# Autodesk Inventor assembly: robot
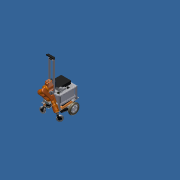
[picture p0: Inventor's stored thumbnail of the model, 180x180]
Saved by Autodesk Inventor 2012 (Build 160160000, 160)
## iProperties
Created: 2012-03-08
Part Number: robot
Document SubType Name: Assembly
Designer: esv
Mass: 169922 g
Surface Area: 87342.5 cm^2
Volume: 147894 cm^3
Density: 1.14894 g/cm^3
Author: esv
## Documents named in this file (28)
- C:\Users\Edward\Documents\masters\CAD\robot.iam
- C:\Users\Edward\Documents\masters\CAD\Frame\frame bracket.ipt
- C:\Users\Edward\Documents\masters\CAD\Invacare\invacare assy.iam
- C:\Users\Edward\Documents\masters\CAD\IRC5\IRC5_Compact.ipt
- C:\Users\Edward\Documents\masters\CAD\Frame\lower side rail.ipt
- C:\Users\Edward\Documents\masters\CAD\Frame\lower front rail.ipt
- C:\Users\Edward\Documents\masters\CAD\Frame\lower vertical rail.ipt
- C:\Users\Edward\Documents\masters\CAD\PC\PC.ipt
- C:\Users\Edward\Documents\masters\CAD\SICK\SICK LMS291.ipt
- C:\Users\Edward\Documents\masters\CAD\Frame\arm rail.ipt
- C:\Users\Edward\Documents\masters\CAD\IRB120\IRB120.iam
- C:\Users\Edward\Documents\masters\CAD\Frame\front upright.ipt
- C:\Users\Edward\Documents\masters\CAD\Kinect\Kinect.ipt
- C:\Users\Edward\Documents\masters\CAD\Frame\front top side rail.ipt
- C:\Users\Edward\Documents\masters\CAD\Frame\aim rail cross brace.ipt
- C:\Users\Edward\Documents\masters\CAD\Frame\back frame plate.ipt
- C:\Users\Edward\Documents\masters\CAD\Frame\front frame plate.ipt
- C:\Users\Edward\Documents\masters\CAD\Frame\top plate.ipt
- C:\Users\Edward\Documents\masters\CAD\Pneumatics\compressor\compressor.iam
- C:\Users\Edward\Documents\masters\CAD\Spike\Spike H.iam
- C:\Users\Edward\Documents\masters\CAD\Breaker\Breaker.iam
- C:\Users\Edward\Documents\masters\CAD\Router\router keepout.ipt
- C:\Users\Edward\Documents\masters\CAD\LIDAR Power Supply\LIDAR PSU.ipt
- C:\Users\Edward\Documents\masters\CAD\Frame\front right plate.ipt
- C:\Users\Edward\Documents\masters\CAD\Frame\front left plate.ipt
- C:\Users\Edward\Documents\masters\CAD\Frame\short frame bracket.ipt
- C:\Users\Edward\Documents\masters\CAD\base plate.iam
- C:\Users\Edward\Documents\masters\CAD\SICK\LIDAR Bracket.ipt
## Components (40 placed, 27 different names)
1. frame bracket:1 — Angle:1, Flush:5, Mate:39, Mate:40, Mate:41, Mate:72, Flush:56, Mate:74
2. frame bracket:4 — Flush:5, Mate:27, Mate:42, Mate:43, Mate:44, Flush:57, Mate:75, Mate:76
3. invacare assy:1 [sub-assembly] — Angle:1, Flush:31, Mate:18, Mate:17, Mate:68, Mate:71, Flush:54, Mate:73, Mate:77, Flush:83
4. IRC5_Compact:1 — Flush:2, Mate:7, Mate:8, Mate:99
5. lower side rail:1 — Flush:9, Flush:12, Flush:14, Flush:76, Mate:108, Mate:113, Flush:84
6. lower side rail:2 — Flush:9, Mate:6, Flush:10, Flush:12, Flush:13, Flush:41, Flush:42, Mate:45, Flush:59, Flush:62, Flush:81
7. lower side rail:3 — Flush:8, Mate:6, Flush:11, Flush:14, Mate:7, Mate:8, Flush:71
8. lower side rail:4 — Flush:8, Flush:10, Flush:11, Flush:13, Mate:79, Angle:3
9. PC:1 — Mate:36, Flush:62, Flush:63
10. SICK LMS291:1 — Insert:8, Insert:9, Mate:118
11. arm rail:1 — Flush:26, Flush:35, Mate:27, Mate:37, Tangent:1, Mate:49, Mate:53
12. arm rail:2 — Flush:26, Flush:35, Mate:30, Mate:50, Flush:49, Flush:50, Mate:84, Flush:65, Mate:115
13. IRB120:1 [sub-assembly] — Tangent:1, Mate:30, Mate:37
14. front upright:1 — Mate:39, Mate:40, Mate:41, Flush:41, Flush:42, Mate:45, Mate:47, Flush:46, Flush:47, Mate:51, Mate:101, Flush:78
15. front upright:2 — Mate:42, Mate:43, Mate:44, Flush:43, Flush:44, Flush:45, Mate:52, Flush:71, Mate:103, Flush:79
16. lower front rail:3 — Mate:47, Flush:43, Mate:112, Mate:114, Flush:84, Mate:115, Mate:116, Mate:117
17. Kinect:1 — Mate:54, Flush:51, Mate:55, Angle:2
18. front top side rail:1 — Flush:46, Flush:47, Mate:50, Mate:51, Flush:55
19. front top side rail:2 — Mate:49, Flush:44, Flush:45, Mate:52, Flush:55, Flush:77
20. aim rail cross brace:1 — Flush:49, Flush:50, Mate:53, Mate:54, Flush:51
21. back frame plate:1 — Mate:68, Flush:54, Flush:82, Insert:7
22. back frame plate:2 — Mate:71, Insert:6
23. front frame plate:1 — Flush:57, Mate:75, Mate:76, Mate:77
24. front frame plate:2 — Mate:72, Flush:56, Mate:73, Mate:74
25. top plate:1 — Mate:79, Flush:59, Mate:36, Mate:80, Flush:63, Mate:81, Insert:1, Insert:2, Insert:3, Mate:82, Insert:4, Insert:5, Flush:64, Flush:77, Mate:102
26. compressor:1 [sub-assembly] — Mate:80, Insert:2, Insert:3
27. Spike H:1 [sub-assembly] — Mate:81, Insert:1
28. Breaker:1 [sub-assembly] — Mate:82, Insert:4, Angle:3, Insert:5
29. router keepout:1 — Flush:64, Mate:83, Mate:84
30. LIDAR PSU:1 — Flush:65, Tangent:5, Tangent:6
31. lower vertical rail:1 — Flush:69, Flush:70, Flush:74, Flush:75, Mate:100, Mate:110, Mate:111
32. lower vertical rail:2 — Flush:69, Flush:70, Mate:99, Mate:104, Mate:105, Mate:106, Mate:107, Mate:108, Flush:81
33. lower front rail:4 — Flush:72, Flush:73, Flush:74, Flush:75, Mate:100
34. lower front rail:5 — Flush:72, Flush:73, Flush:76, Mate:107, Mate:109
35. front right plate:1 — Mate:101, Flush:78, Mate:102, Flush:80, Tangent:5, Tangent:6
36. front left plate:1 — Mate:103, Flush:79, Flush:80
37. short frame bracket:1 — Mate:104, Mate:105, Insert:6, Mate:106, Mate:109
38. short frame bracket:2 — Mate:110, Mate:111, Flush:82, Insert:7, Flush:83
39. base plate:1 [sub-assembly] — Mate:112, Mate:113, Mate:114
40. LIDAR Bracket:1 — Insert:8, Insert:9, Mate:116, Mate:117
## Relationships (122: Mate 59, Flush 48, Insert 9, Angle 3, Tangent 3)
- Flush:2 (-225 mm): IRC5_Compact:1
- Angle:1 (0 deg): frame bracket:1 ↔ invacare assy:1
- Flush:5: frame bracket:1 ↔ frame bracket:4
- Flush:8: lower side rail:3 ↔ lower side rail:4
- Flush:9: lower side rail:1 ↔ lower side rail:2
- Mate:6 (450.85 mm): lower side rail:2 ↔ lower side rail:3
- Flush:10: lower side rail:2 ↔ lower side rail:4
- Flush:11: lower side rail:3 ↔ lower side rail:4
- Flush:12: lower side rail:1 ↔ lower side rail:2
- Flush:13: lower side rail:2 ↔ lower side rail:4
- Flush:14: lower side rail:1 ↔ lower side rail:3
- Mate:7: IRC5_Compact:1 ↔ lower side rail:3
- Mate:8 (6.35 mm): IRC5_Compact:1 ↔ lower side rail:3
- Flush:31: invacare assy:1
- Mate:17: invacare assy:1
- Mate:18: invacare assy:1
- Flush:26: arm rail:1 ↔ arm rail:2
- Flush:35: arm rail:1 ↔ arm rail:2
- Mate:27: frame bracket:4 ↔ arm rail:1
- Tangent:1: arm rail:1 ↔ IRB120:1
- Mate:30: arm rail:2 ↔ IRB120:1
- Mate:37 (-609.6 mm): arm rail:1 ↔ IRB120:1
- Mate:36: PC:1 ↔ top plate:1
- Flush:40 (-368.3 mm)
- Mate:39: frame bracket:1 ↔ front upright:1
- Mate:40: frame bracket:1 ↔ front upright:1
- Mate:41: frame bracket:1 ↔ front upright:1
- Mate:42: frame bracket:4 ↔ front upright:2
- Mate:43: frame bracket:4 ↔ front upright:2
- Mate:44: frame bracket:4 ↔ front upright:2
- Flush:41: lower side rail:2 ↔ front upright:1
- Flush:42: lower side rail:2 ↔ front upright:1
- Mate:45: lower side rail:2 ↔ front upright:1
- Mate:47: front upright:1 ↔ lower front rail:3
- Flush:43: front upright:2 ↔ lower front rail:3
- Mate:49: arm rail:1 ↔ front top side rail:2
- Flush:44: front upright:2 ↔ front top side rail:2
- Flush:45: front upright:2 ↔ front top side rail:2
- Flush:46: front upright:1 ↔ front top side rail:1
- Flush:47: front upright:1 ↔ front top side rail:1
- Mate:50: arm rail:2 ↔ front top side rail:1
- Mate:51: front upright:1 ↔ front top side rail:1
- Mate:52: front upright:2 ↔ front top side rail:2
- Flush:49: arm rail:2 ↔ aim rail cross brace:1
- Flush:50: arm rail:2 ↔ aim rail cross brace:1
- Mate:53: arm rail:1 ↔ aim rail cross brace:1
- Mate:54: Kinect:1 ↔ aim rail cross brace:1
- Flush:51: Kinect:1 ↔ aim rail cross brace:1
- Mate:55: Kinect:1
- Angle:2 (0 deg): Kinect:1
- Mate:56
- Mate:68: invacare assy:1 ↔ back frame plate:1
- Mate:71: invacare assy:1 ↔ back frame plate:2
- Flush:54: invacare assy:1 ↔ back frame plate:1
- Flush:55: front top side rail:1 ↔ front top side rail:2
- Mate:72: frame bracket:1 ↔ front frame plate:2
- Flush:56: frame bracket:1 ↔ front frame plate:2
- Mate:73: invacare assy:1 ↔ front frame plate:2
- Mate:74: frame bracket:1 ↔ front frame plate:2
- Flush:57: frame bracket:4 ↔ front frame plate:1
- Mate:75: frame bracket:4 ↔ front frame plate:1
- Mate:76: frame bracket:4 ↔ front frame plate:1
- Mate:77: invacare assy:1 ↔ front frame plate:1
- Mate:79: lower side rail:4 ↔ top plate:1
- Flush:59: lower side rail:2 ↔ top plate:1
- Mate:80: top plate:1 ↔ compressor:1
- Flush:62 (50.8 mm): lower side rail:2 ↔ PC:1
- Flush:63 (-50.8 mm): PC:1 ↔ top plate:1
- Mate:81: top plate:1 ↔ Spike H:1
- Insert:1: top plate:1 ↔ Spike H:1
- Insert:2: top plate:1 ↔ compressor:1
- Insert:3: top plate:1 ↔ compressor:1
- Mate:82: top plate:1 ↔ Breaker:1
- Insert:4: top plate:1 ↔ Breaker:1
- Angle:3 (0 deg): lower side rail:4 ↔ Breaker:1
- Insert:5: top plate:1 ↔ Breaker:1
- Flush:64 (-304.8 mm): top plate:1 ↔ router keepout:1
- Mate:83: router keepout:1
- Mate:84: arm rail:2 ↔ router keepout:1
- Flush:65: arm rail:2 ↔ LIDAR PSU:1
- Flush:69: lower vertical rail:1 ↔ lower vertical rail:2
- Flush:70: lower vertical rail:1 ↔ lower vertical rail:2
- Flush:71: lower side rail:3 ↔ front upright:2
- Mate:99: IRC5_Compact:1 ↔ lower vertical rail:2
- Flush:72: lower front rail:4 ↔ lower front rail:5
- Flush:73: lower front rail:4 ↔ lower front rail:5
- Flush:74: lower vertical rail:1 ↔ lower front rail:4
- Flush:75: lower vertical rail:1 ↔ lower front rail:4
- Mate:100: lower vertical rail:1 ↔ lower front rail:4
- Flush:76: lower side rail:1 ↔ lower front rail:5
- Flush:77: front top side rail:2 ↔ top plate:1
- Mate:101: front upright:1 ↔ front right plate:1
- Flush:78: front upright:1 ↔ front right plate:1
- Mate:102: top plate:1 ↔ front right plate:1
- Mate:103: front upright:2 ↔ front left plate:1
- Flush:79: front upright:2 ↔ front left plate:1
- Flush:80: front right plate:1 ↔ front left plate:1
- Tangent:5: LIDAR PSU:1 ↔ front right plate:1
- Tangent:6: LIDAR PSU:1 ↔ front right plate:1
- Mate:104: lower vertical rail:2 ↔ short frame bracket:1
- Mate:105: lower vertical rail:2 ↔ short frame bracket:1
- Insert:6: back frame plate:2 ↔ short frame bracket:1
- Mate:106: lower vertical rail:2 ↔ short frame bracket:1
- Mate:107: lower vertical rail:2 ↔ lower front rail:5
- Mate:108: lower side rail:1 ↔ lower vertical rail:2
- Flush:81: lower side rail:2 ↔ lower vertical rail:2
- Mate:109: lower front rail:5 ↔ short frame bracket:1
- Mate:110: lower vertical rail:1 ↔ short frame bracket:2
- Mate:111: lower vertical rail:1 ↔ short frame bracket:2
- Flush:82: back frame plate:1 ↔ short frame bracket:2
- Insert:7: back frame plate:1 ↔ short frame bracket:2
- Flush:83: invacare assy:1 ↔ short frame bracket:2
- Mate:112: lower front rail:3 ↔ base plate:1
- Mate:113: lower side rail:1 ↔ base plate:1
- Mate:114: lower front rail:3 ↔ base plate:1
- Flush:84: lower side rail:1 ↔ lower front rail:3
- Mate:115: arm rail:2 ↔ lower front rail:3
- Insert:8: SICK LMS291:1 ↔ LIDAR Bracket:1
- Insert:9: SICK LMS291:1 ↔ LIDAR Bracket:1
- Mate:116: lower front rail:3 ↔ LIDAR Bracket:1
- Mate:117: lower front rail:3 ↔ LIDAR Bracket:1
- Mate:118: SICK LMS291:1
